# Autodesk Inventor assembly: SYSTEM-FLANGE
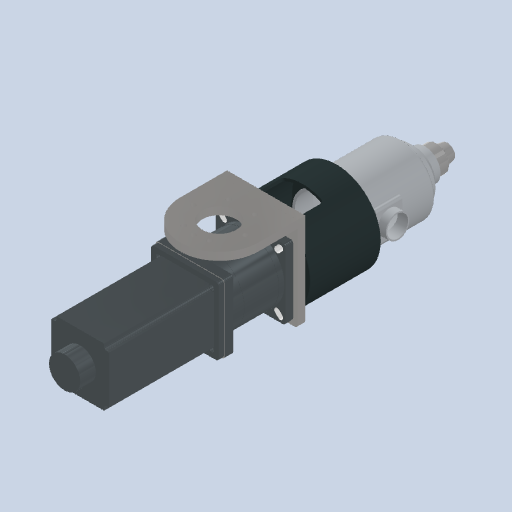
[picture p0: Inventor's stored thumbnail of the model, 512x512]
Saved by Autodesk Inventor 2025.3 (Build 293356030, 356C)
## iProperties
Created: 2025-11-27
Part Number: SYSTEM-FLANGE
Document SubType Name: Assembly
Designer: lstk1ng
Author: lstk1ng
## Documents named in this file (8)
- C:\Users\lstk1ng\Documents\UPC\UPC-10\PROYECTO MECATRONICO 1\DISEÑO MECANICO\SYSTEM-FLANGE.iam
- C:\Users\lstk1ng\Documents\UPC\UPC-10\PROYECTO MECATRONICO 1\DISEÑO MECANICO\SYSTEM-FLANGE-K60.ipt
- C:\Users\lstk1ng\Documents\UPC\UPC-10\PROYECTO MECATRONICO 1\DISEÑO MECANICO\SYSTEM-FLANGE-LOWER.ipt
- C:\Users\lstk1ng\Documents\UPC\UPC-10\PROYECTO MECATRONICO 1\DISEÑO MECANICO\COMPONENTS\PX130-GEARBOX.ipt
- C:\Users\lstk1ng\Documents\UPC\UPC-10\PROYECTO MECATRONICO 1\DISEÑO MECANICO\COMPONENTS\SERVOMOTOR-2.3KWv1.ipt
- C:\Users\lstk1ng\Documents\UPC\UPC-10\PROYECTO MECATRONICO 1\DISEÑO MECANICO\UPPER-NOZZLEv3.1.ipt
- C:\Users\lstk1ng\Documents\UPC\UPC-10\PROYECTO MECATRONICO 1\DISEÑO MECANICO\LOWER-NOZZLEv2.ipt
- C:\Users\lstk1ng\Documents\UPC\UPC-10\PROYECTO MECATRONICO 1\DISEÑO MECANICO\NOZZLE-EXTRUSOR.ipt
## Components (7 placed, 7 different names)
1. SYSTEM-FLANGE-K60:1 — Mate:1, Mate:2, Mate:3
2. SYSTEM-FLANGE-LOWER:1 — Mate:1, Mate:2, Mate:3, Mate:4, Mate:7, Mate:8, Mate:11
3. PX130-GEARBOX:1 — Mate:4, Mate:5, Mate:6, Mate:7, Mate:8, Mate:9, Mate:10
4. SERVOMOTOR-2.3KWv1:1 — Mate:5, Mate:6, Mate:9
5. UPPER-NOZZLEv3.1:1 — Mate:10, Mate:11, Insert:1
6. LOWER-NOZZLEv2:1 — Insert:1, Insert:2
7. NOZZLE-EXTRUSOR:1 — Insert:2
## Relationships (13: Mate 11, Insert 2)
- Mate:1: SYSTEM-FLANGE-K60:1 ↔ SYSTEM-FLANGE-LOWER:1
- Mate:2: SYSTEM-FLANGE-K60:1 ↔ SYSTEM-FLANGE-LOWER:1
- Mate:3: SYSTEM-FLANGE-K60:1 ↔ SYSTEM-FLANGE-LOWER:1
- Mate:4: SYSTEM-FLANGE-LOWER:1 ↔ PX130-GEARBOX:1
- Mate:5: PX130-GEARBOX:1 ↔ SERVOMOTOR-2.3KWv1:1
- Mate:6: PX130-GEARBOX:1 ↔ SERVOMOTOR-2.3KWv1:1
- Mate:7: SYSTEM-FLANGE-LOWER:1 ↔ PX130-GEARBOX:1
- Mate:8: SYSTEM-FLANGE-LOWER:1 ↔ PX130-GEARBOX:1
- Mate:9: PX130-GEARBOX:1 ↔ SERVOMOTOR-2.3KWv1:1
- Mate:10: PX130-GEARBOX:1 ↔ UPPER-NOZZLEv3.1:1
- Mate:11: SYSTEM-FLANGE-LOWER:1 ↔ UPPER-NOZZLEv3.1:1
- Insert:1: UPPER-NOZZLEv3.1:1 ↔ LOWER-NOZZLEv2:1
- Insert:2: LOWER-NOZZLEv2:1 ↔ NOZZLE-EXTRUSOR:1
